# Autodesk Inventor assembly: Scoreboard
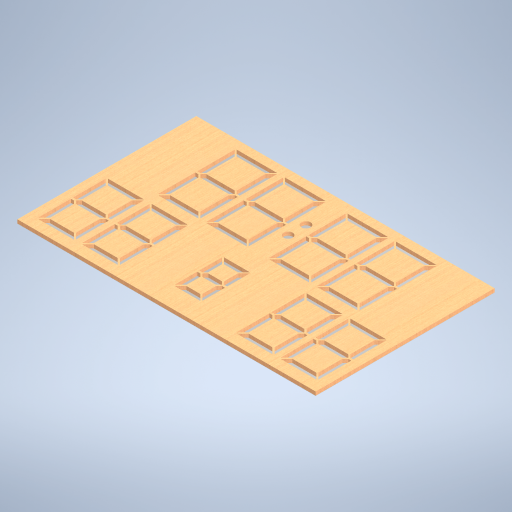
[picture p0: Inventor's stored thumbnail of the model, 512x512]
Saved by Autodesk Inventor 2024 (Build 280153000, 153)
## iProperties
Created: 2024-02-15
Part Number: Scoreboard
Document SubType Name: Assembly
Designer: haniv
Author: haniv
## Documents named in this file (3)
- C:\Users\haniv\Desktop\Unterlagen\Projekte\7_Segment_Anzeige\ScoreDisplay\CAD\Scoreboard.iam
- C:\Users\haniv\Desktop\Unterlagen\Projekte\7_Segment_Anzeige\ScoreDisplay\CAD\Components\Aluminium_Grundplatte.ipt
- C:\Users\haniv\Desktop\Unterlagen\Projekte\7_Segment_Anzeige\ScoreDisplay\CAD\Components\MDF_Anzeige.ipt
## Components (2 placed, 2 different names)
1. Aluminium_Grundplatte:1 — Passend:1, Fluchtend:1, Fluchtend:2
2. MDF_Anzeige:1 — Passend:1, Fluchtend:1, Fluchtend:2
## Relationships (3: Flush 2, Mate 1)
- Passend:1 [Mate]: Aluminium_Grundplatte:1 ↔ MDF_Anzeige:1
- Fluchtend:1 [Flush]: Aluminium_Grundplatte:1 ↔ MDF_Anzeige:1
- Fluchtend:2 [Flush]: Aluminium_Grundplatte:1 ↔ MDF_Anzeige:1
